# Autodesk Inventor assembly: Plow_Assembly
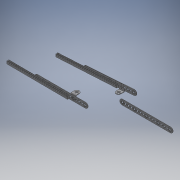
[picture p0: Inventor's stored thumbnail of the model, 180x180]
Saved by Autodesk Inventor 2016 (Build 200138000, 138)
## iProperties
Created: 2015-10-23
Part Number: Plow_Assembly
Document SubType Name: Assembly
Designer: Delta
Author: Delta
## Documents named in this file (4)
- C:\Robotics\2015-16_CAD\custom cad parts\Plow_Assembly.iam
- C:\Robotics\2015-16_CAD\COTSParts\Tetrix\Tetrix bracket - angle.ipt
- C:\Robotics\2015-16_CAD\COTSParts\Actobotics\585 parts\585398.ipt
- C:\Robotics\2015-16_CAD\custom cad parts\Tetrix Max Flat 288mm.ipt
## Components (7 placed, 3 different names)
1. Tetrix bracket - angle:1 — Insert:1
2. Tetrix bracket - angle:2 — Insert:2
3. 585398:1 — Insert:3
4. 585398:2 — Insert:4
5. Tetrix Max Flat 288mm:1 — Insert:2, Insert:4
6. Tetrix Max Flat 288mm:2 — Insert:1, Insert:3
7. Tetrix Max Flat 288mm:3
## Relationships (4: Insert 4)
- Insert:1: Tetrix bracket - angle:1 ↔ Tetrix Max Flat 288mm:2
- Insert:2: Tetrix bracket - angle:2 ↔ Tetrix Max Flat 288mm:1
- Insert:3: 585398:1 ↔ Tetrix Max Flat 288mm:2
- Insert:4: 585398:2 ↔ Tetrix Max Flat 288mm:1
